# Autodesk Inventor assembly: Quick Release Assy
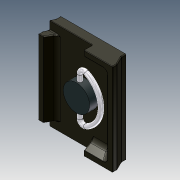
[picture p0: Inventor's stored thumbnail of the model, 180x180]
Saved by Autodesk Inventor 2011 (Build 150239000, 239)
## iProperties
Created: 2012-10-13
Part Number: Quick Release Assy
Document SubType Name: Assembly
Designer: Lance
Author: Lance
## Documents named in this file (5)
- C:\Inventor Projects\MPX0032 - Projector Accessories\Manfrotto 494RC2 - Tripod Head\Quick Release Assy.iam
- C:\Inventor Projects\MPX0032 - Projector Accessories\Manfrotto 494RC2 - Tripod Head\Quick Release Mounting.ipt
- C:\Inventor Projects\MPX0032 - Projector Accessories\Manfrotto 494RC2 - Tripod Head\Thumb Screw Assy.iam
- C:\Users\Lance\Documents\Inventor\Content Center Files\R2011\en-US\IS 3075-3\IS 3075-3 - 3.2 - 0.6 - 4.ipt
- C:\Inventor Projects\MPX0032 - Projector Accessories\Manfrotto 494RC2 - Tripod Head\Quick Release Rubber Pad.ipt
## Components (4 placed, 4 different names)
1. Quick Release Mounting:1 — Insert:1, Angle:1, Mate:3, Mate:4, Angle:2
2. Thumb Screw Assy:1 [sub-assembly] — Insert:1, Angle:1, Mate:1, Mate:2
3. IS 3075-3 3.2:1 — Mate:1, Mate:2, Flush:1
4. Quick Release Rubber Pad:1 — Mate:3, Mate:4, Angle:2
## Relationships (8: Mate 4, Angle 2, Insert 1, Flush 1)
- Insert:1: Quick Release Mounting:1 ↔ Thumb Screw Assy:1
- Angle:1 (180 deg): Quick Release Mounting:1 ↔ Thumb Screw Assy:1
- Mate:1: Thumb Screw Assy:1 ↔ IS 3075-3 3.2:1
- Mate:2: Thumb Screw Assy:1 ↔ IS 3075-3 3.2:1
- Flush:1: IS 3075-3 3.2:1
- Mate:3: Quick Release Mounting:1 ↔ Quick Release Rubber Pad:1
- Mate:4: Quick Release Mounting:1 ↔ Quick Release Rubber Pad:1
- Angle:2 (180 deg): Quick Release Mounting:1 ↔ Quick Release Rubber Pad:1
